# Autodesk Inventor assembly: Male to Male
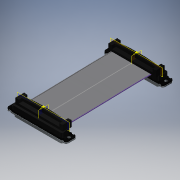
[picture p0: Inventor's stored thumbnail of the model, 180x180]
Saved by Autodesk Inventor 2019 (Build 230136000, 136)
## iProperties
Created: 2019-02-06
Part Number: Male to Male
Document SubType Name: Assembly
Designer: Serge
Author: Serge
## Documents named in this file (4)
- C:\Users\Serge\Desktop\Ribbon Cable\Male to Male.iam
- C:\Users\Serge\Desktop\Ribbon Cable\Ribbon Cable Male.iam
- C:\Users\Serge\Desktop\Ribbon Cable\Ribbon Cable Male Both Directions.iam
- C:\Users\Serge\Desktop\Ribbon Cable\Male to Male\AIP\Cable and Harness\Male to Male.Harness2.iam
## Components (3 placed, 3 different names)
1. Ribbon Cable Male:1 [sub-assembly] — Mate:2, Flush:2
2. Ribbon Cable Male Both Directions:3 [sub-assembly] — Mate:2, Flush:2
3. Harness2 [sub-assembly]
## Relationships (2: Mate 1, Flush 1)
- Mate:2 (100 mm): Ribbon Cable Male:1 ↔ Ribbon Cable Male Both Directions:3
- Flush:2: Ribbon Cable Male:1 ↔ Ribbon Cable Male Both Directions:3
